# Autodesk Inventor assembly: final assembly 1
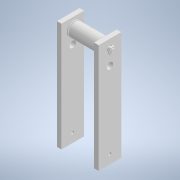
[picture p0: Inventor's stored thumbnail of the model, 180x180]
Saved by Autodesk Inventor 2022 (Build 260153000, 153)
## iProperties
Created: 2022-06-16
Part Number: final assembly 1
Document SubType Name: Assembly
Designer: chait
Author: chait
## Documents named in this file (3)
- C:\Users\chait\Documents\final assembly 1.iam
- C:\Users\chait\Documents\new assembly.iam
- C:\Users\chait\Documents\Bolt 5mm.ipt
## Components (3 placed, 2 different names)
1. new assembly:1 [sub-assembly]
2. new assembly:2 [sub-assembly] — Insert:1
3. Bolt 5mm:2 — Insert:1
## Relationships (1: Insert 1)
- Insert:1 (1 mm): new assembly:2 ↔ Bolt 5mm:2
